# Autodesk Inventor assembly: luer-straight-adapter
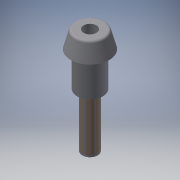
[picture p0: Inventor's stored thumbnail of the model, 180x180]
Saved by Autodesk Inventor 2016 (Build 200138000, 138)
## iProperties
Created: 2016-04-27
Part Number: luer-straight-adapter
Document SubType Name: Weldment
Designer: GentnerLab
Weld Material: Welded Aluminum-6061
Author: GentnerLab
## Documents named in this file (3)
- C:\Users\GentnerLab\Documents\GentnerLabSTL\luer-straight-adapter.iam
- C:\Users\GentnerLab\Documents\Inventor\Parts\luer_fit.ipt
- C:\Users\GentnerLab\Documents\Inventor\Parts\straight_fit.ipt
## Components (2 placed, 2 different names)
1. luer_fit:1 — Rigid:1
2. straight_fit:2 — Rigid:1
## Relationships (1: WeldJoint 1)
- Rigid:1 [WeldJoint]: luer_fit:1 ↔ straight_fit:2
